# Autodesk Inventor assembly: sekkeiseisakuron
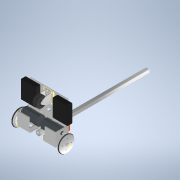
[picture p0: Inventor's stored thumbnail of the model, 180x180]
Saved by Autodesk Inventor 2022 (Build 260153000, 153)
## iProperties
Created: 2021-10-16
Part Number: sekkeiseisakuron
Document SubType Name: Assembly
Designer: gilte
Author: gilte
## Documents named in this file (21)
- C:\Users\shiok\Documents\GitHub\University\minakatalab\shacho\sekkeiseisakuron.0001.iam
- C:\Users\shiok\Documents\GitHub\University\minakatalab\shacho\RD002_フレーム.ipt
- C:\Users\shiok\Documents\GitHub\University\minakatalab\shacho\RD006_ギヤボックス左.ipt
- C:\Users\shiok\Documents\GitHub\University\minakatalab\shacho\RD007_ギヤボックス右.ipt
- C:\Users\shiok\Documents\GitHub\University\minakatalab\shacho\RD005_ペンホルダ.ipt
- C:\Users\shiok\Documents\GitHub\University\minakatalab\shacho\RD014_ストッパ.ipt
- C:\Users\shiok\Documents\GitHub\University\minakatalab\shacho\RD015_シャフト.ipt
- C:\Users\shiok\Documents\GitHub\University\minakatalab\shacho\RD008_モータ(DMN29).ipt
- C:\Users\shiok\Documents\GitHub\University\minakatalab\shacho\RD009_ギアDS0.5-12.ipt
- C:\Users\shiok\Documents\GitHub\University\minakatalab\shacho\RD020_ワッシャ.ipt
- C:\Users\shiok\Documents\GitHub\University\minakatalab\shacho\RD019_ブッシュ80F-0305改.ipt
- C:\Users\shiok\Documents\GitHub\University\minakatalab\shacho\RD010_ギアDS0.5-80.ipt
- C:\Users\shiok\Documents\GitHub\University\minakatalab\shacho\RD011_ギア用ブッシュ.ipt
- C:\Users\shiok\Documents\GitHub\University\minakatalab\shacho\RD018_ブッシュ80F-0305.ipt
- C:\Users\shiok\Documents\GitHub\University\minakatalab\shacho\RD012_ホイール.ipt
- C:\Users\shiok\Documents\GitHub\University\minakatalab\shacho\RD013_オーリング.ipt
- C:\Users\shiok\Documents\GitHub\University\minakatalab\shacho\additionalhand.iam
- C:\Users\shiok\Documents\GitHub\University\minakatalab\shacho\RD004_スペーサ改.ipt
- C:\Users\shiok\Documents\GitHub\University\minakatalab\shacho\cast.iam
- C:\Users\shiok\Documents\GitHub\University\minakatalab\shacho\batterybox.ipt
- C:\Users\shiok\Documents\GitHub\University\minakatalab\shacho\batterybox_MIR.ipt
## Components (33 placed, 20 different names)
1. RD002_フレーム:1 — 挿入:9, 挿入:10, 挿入:28, 挿入:29, 挿入:30, メイト:3, メイト:4, メイト:5, メイト:6, メイト:7, メイト:8, フラッシュ:1, メイト:10, メイト:15, メイト:17
2. RD005_ペンホルダ:1 — 挿入:9, 挿入:10
3. RD014_ストッパ:2 — 挿入:47
4. RD014_ストッパ:4 — 挿入:48
5. RD010_ギアDS0.5-80:1 — 挿入:25
6. RD011_ギア用ブッシュ:1 — 挿入:25, 挿入:42, 挿入:45
7. RD006_ギヤボックス左:1 — 挿入:28, 挿入:29, 挿入:32, 挿入:33, 挿入:36, 挿入:51, 挿入:52
8. RD007_ギヤボックス右:1 — 挿入:30, 挿入:31, 挿入:37, 挿入:49, 挿入:50, メイト:9, メイト:10
9. RD014_ストッパ:5 — 挿入:31, 挿入:35
10. RD014_ストッパ:6 — 挿入:32, 挿入:33, 挿入:34
11. RD015_シャフト:1 — 挿入:34
12. RD015_シャフト:2 — 挿入:35
13. RD020_ワッシャ:1 — 挿入:36, 挿入:39
14. RD020_ワッシャ:2 — 挿入:37, 挿入:38
15. RD019_ブッシュ80F-0305改:1 — 挿入:38, 挿入:42
16. RD019_ブッシュ80F-0305改:2 — 挿入:39, 挿入:41
17. RD010_ギアDS0.5-80:2 — 挿入:40
18. RD011_ギア用ブッシュ:2 — 挿入:40, 挿入:41, 挿入:46
19. RD018_ブッシュ80F-0305:1 — 挿入:44, 挿入:46, 挿入:47
20. RD018_ブッシュ80F-0305:2 — 挿入:43, 挿入:45, 挿入:48
21. RD012_ホイール:1 — 挿入:43, メイト:1, 正接:1
22. RD012_ホイール:2 — 挿入:44, メイト:2, 正接:2
23. RD008_モータ(DMN29):1 — 挿入:51, 挿入:52, 挿入:53
24. RD008_モータ(DMN29):2 — 挿入:49, 挿入:50, 挿入:54
25. RD009_ギアDS0.5-12:1 — 挿入:54
26. RD009_ギアDS0.5-12:2 — 挿入:53
27. RD013_オーリング:1 — メイト:1, 正接:1
28. RD013_オーリング:2 — メイト:2, 正接:2
29. additionalhand:1 [sub-assembly] — メイト:3, メイト:4, メイト:5, メイト:11
30. RD004_スペーサ改:1 — メイト:6, メイト:7, メイト:8, メイト:12, メイト:13, メイト:14
31. cast:1 [sub-assembly] — メイト:12, メイト:13, メイト:14
32. batterybox:1 — メイト:15, メイト:17
33. batterybox_MIR:1
## Relationships (49: Insert 30, Mate 16, Tangent 2, Flush 1)
- 挿入:9 [Insert]: RD002_フレーム:1 ↔ RD005_ペンホルダ:1
- 挿入:10 [Insert]: RD002_フレーム:1 ↔ RD005_ペンホルダ:1
- 挿入:25 [Insert]: RD010_ギアDS0.5-80:1 ↔ RD011_ギア用ブッシュ:1
- 挿入:28 [Insert]: RD002_フレーム:1 ↔ RD006_ギヤボックス左:1
- 挿入:29 [Insert]: RD002_フレーム:1 ↔ RD006_ギヤボックス左:1
- 挿入:30 [Insert]: RD002_フレーム:1 ↔ RD007_ギヤボックス右:1
- 挿入:31 [Insert]: RD007_ギヤボックス右:1 ↔ RD014_ストッパ:5
- 挿入:32 [Insert]: RD006_ギヤボックス左:1 ↔ RD014_ストッパ:6
- 挿入:33 [Insert]: RD006_ギヤボックス左:1 ↔ RD014_ストッパ:6
- 挿入:34 [Insert]: RD014_ストッパ:6 ↔ RD015_シャフト:1
- 挿入:35 [Insert]: RD014_ストッパ:5 ↔ RD015_シャフト:2
- 挿入:36 [Insert]: RD006_ギヤボックス左:1 ↔ RD020_ワッシャ:1
- 挿入:37 [Insert]: RD007_ギヤボックス右:1 ↔ RD020_ワッシャ:2
- 挿入:38 [Insert]: RD020_ワッシャ:2 ↔ RD019_ブッシュ80F-0305改:1
- 挿入:39 [Insert]: RD020_ワッシャ:1 ↔ RD019_ブッシュ80F-0305改:2
- 挿入:40 [Insert]: RD010_ギアDS0.5-80:2 ↔ RD011_ギア用ブッシュ:2
- 挿入:41 [Insert]: RD019_ブッシュ80F-0305改:2 ↔ RD011_ギア用ブッシュ:2
- 挿入:42 [Insert]: RD011_ギア用ブッシュ:1 ↔ RD019_ブッシュ80F-0305改:1
- 挿入:43 [Insert]: RD018_ブッシュ80F-0305:2 ↔ RD012_ホイール:1
- 挿入:44 [Insert]: RD018_ブッシュ80F-0305:1 ↔ RD012_ホイール:2
- 挿入:45 [Insert]: RD011_ギア用ブッシュ:1 ↔ RD018_ブッシュ80F-0305:2
- 挿入:46 [Insert]: RD011_ギア用ブッシュ:2 ↔ RD018_ブッシュ80F-0305:1
- 挿入:47 [Insert]: RD014_ストッパ:2 ↔ RD018_ブッシュ80F-0305:1
- 挿入:48 [Insert]: RD014_ストッパ:4 ↔ RD018_ブッシュ80F-0305:2
- 挿入:49 [Insert]: RD007_ギヤボックス右:1 ↔ RD008_モータ(DMN29):2
- 挿入:50 [Insert]: RD007_ギヤボックス右:1 ↔ RD008_モータ(DMN29):2
- 挿入:51 [Insert]: RD006_ギヤボックス左:1 ↔ RD008_モータ(DMN29):1
- 挿入:52 [Insert]: RD006_ギヤボックス左:1 ↔ RD008_モータ(DMN29):1
- 挿入:53 [Insert]: RD008_モータ(DMN29):1 ↔ RD009_ギアDS0.5-12:2
- 挿入:54 [Insert]: RD008_モータ(DMN29):2 ↔ RD009_ギアDS0.5-12:1
- メイト:1 [Mate]: RD012_ホイール:1 ↔ RD013_オーリング:1
- 正接:1 [Tangent]: RD012_ホイール:1 ↔ RD013_オーリング:1
- メイト:2 [Mate]: RD012_ホイール:2 ↔ RD013_オーリング:2
- 正接:2 [Tangent]: RD012_ホイール:2 ↔ RD013_オーリング:2
- メイト:3 [Mate]: RD002_フレーム:1 ↔ additionalhand:1
- メイト:4 [Mate]: RD002_フレーム:1 ↔ additionalhand:1
- メイト:5 [Mate]: RD002_フレーム:1 ↔ additionalhand:1
- メイト:6 [Mate]: RD002_フレーム:1 ↔ RD004_スペーサ改:1
- メイト:7 [Mate]: RD002_フレーム:1 ↔ RD004_スペーサ改:1
- メイト:8 [Mate]: RD002_フレーム:1 ↔ RD004_スペーサ改:1
- メイト:9 [Mate]: RD007_ギヤボックス右:1
- フラッシュ:1 [Flush]: RD002_フレーム:1
- メイト:10 [Mate]: RD002_フレーム:1 ↔ RD007_ギヤボックス右:1
- メイト:11 [Mate]: additionalhand:1
- メイト:12 [Mate]: RD004_スペーサ改:1 ↔ cast:1
- メイト:13 [Mate]: RD004_スペーサ改:1 ↔ cast:1
- メイト:14 [Mate]: RD004_スペーサ改:1 ↔ cast:1
- メイト:15 [Mate]: RD002_フレーム:1 ↔ batterybox:1
- メイト:17 [Mate]: RD002_フレーム:1 ↔ batterybox:1
